# Autodesk Inventor assembly: cradleAssembly
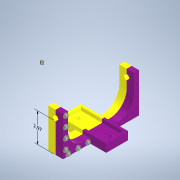
[picture p0: Inventor's stored thumbnail of the model, 180x180]
Saved by Autodesk Inventor 2022 (Build 260153070, 153G)
## iProperties
Created: 2021-06-29
Part Number: cradleAssembly
Document SubType Name: Assembly
Designer: robst
Author: robst
## Documents named in this file (6)
- C:\git\CAD-Development\robSteele\ShapeWays\TelescopeProjects\TelescopeMountNov2020\cradleAssembly.iam
- C:\git\CAD-Development\robSteele\ShapeWays\TelescopeProjects\TelescopeMountNov2020\connectorToTubeBrackeCradlePrintBack.ipt
- C:\git\CAD-Development\robSteele\ShapeWays\TelescopeProjects\TelescopeMountNov2020\connectorToTubeBrackeCradlePrintFront.ipt
- C:\Users\robst\Documents\Inventor\Content Center Files\R2021\en-US\ANSI B18.22.1\ANSI B18.22.1 - No. 10 - Type A.ipt
- C:\Users\robst\Documents\Inventor\Content Center Files\R2021\en-US\ASME B18.21.1(10)\ASME B18.21.1 - No.10(2).ipt
- C:\Users\robst\Documents\Inventor\Content Center Files\R2021\en-US\ANSI B18.6.2(08)\ANSI B18.6.2 - 10-32 UNF - 1.75(17).ipt
## Components (23 placed, 5 different names)
1. connectorToTubeBrackeCradlePrintBack:1 — Mate:1, Flush:1, Flush:2
2. connectorToTubeBrackeCradlePrintFront:1 — Mate:1, Flush:1, Flush:2, Mate:2, Mate:3, Mate:4, Mate:5, Mate:6, Mate:7, Mate:8, Mate:9, Mate:10, Mate:11, Mate:12, Mate:13, Mate:14, Mate:15
3. Plain Washer (Inch) No. 10 - Type A:1 — Mate:2, Mate:3, Insert:1
4. Regular Helical Spring Lock Washer (Inch) No.10:1 — Insert:1, Insert:8
5. Slotted Round Head Cap Screw - Inch No. 10 - 32 - 1 3/4:1 — Insert:8
6. Plain Washer (Inch) No. 10 - Type A:2 — Mate:4, Mate:5, Insert:2
7. Plain Washer (Inch) No. 10 - Type A:3 — Mate:6, Mate:7, Insert:3
8. Plain Washer (Inch) No. 10 - Type A:4 — Mate:8, Mate:9, Insert:4
9. Plain Washer (Inch) No. 10 - Type A:5 — Mate:10, Mate:11, Insert:5
10. Plain Washer (Inch) No. 10 - Type A:6 — Mate:12, Mate:13, Insert:6
11. Plain Washer (Inch) No. 10 - Type A:7 — Mate:14, Mate:15, Insert:7
12. Regular Helical Spring Lock Washer (Inch) No.10:2 — Insert:2, Insert:9
13. Regular Helical Spring Lock Washer (Inch) No.10:3 — Insert:3, Insert:10
14. Regular Helical Spring Lock Washer (Inch) No.10:4 — Insert:4, Insert:11
15. Regular Helical Spring Lock Washer (Inch) No.10:5 — Insert:5, Insert:12
16. Regular Helical Spring Lock Washer (Inch) No.10:6 — Insert:6, Insert:13
17. Regular Helical Spring Lock Washer (Inch) No.10:7 — Insert:7, Insert:14
18. Slotted Round Head Cap Screw - Inch No. 10 - 32 - 1 3/4:2 — Insert:9
19. Slotted Round Head Cap Screw - Inch No. 10 - 32 - 1 3/4:3 — Insert:10
20. Slotted Round Head Cap Screw - Inch No. 10 - 32 - 1 3/4:4 — Insert:11
21. Slotted Round Head Cap Screw - Inch No. 10 - 32 - 1 3/4:5 — Insert:12
22. Slotted Round Head Cap Screw - Inch No. 10 - 32 - 1 3/4:6 — Insert:13
23. Slotted Round Head Cap Screw - Inch No. 10 - 32 - 1 3/4:7 — Insert:14
## Relationships (31: Mate 15, Insert 14, Flush 2)
- Mate:1: connectorToTubeBrackeCradlePrintBack:1 ↔ connectorToTubeBrackeCradlePrintFront:1
- Flush:1: connectorToTubeBrackeCradlePrintBack:1 ↔ connectorToTubeBrackeCradlePrintFront:1
- Flush:2: connectorToTubeBrackeCradlePrintBack:1 ↔ connectorToTubeBrackeCradlePrintFront:1
- Mate:2: connectorToTubeBrackeCradlePrintFront:1 ↔ Plain Washer (Inch) No. 10 - Type A:1
- Mate:3: connectorToTubeBrackeCradlePrintFront:1 ↔ Plain Washer (Inch) No. 10 - Type A:1
- Mate:4: connectorToTubeBrackeCradlePrintFront:1 ↔ Plain Washer (Inch) No. 10 - Type A:2
- Mate:5: connectorToTubeBrackeCradlePrintFront:1 ↔ Plain Washer (Inch) No. 10 - Type A:2
- Mate:6: connectorToTubeBrackeCradlePrintFront:1 ↔ Plain Washer (Inch) No. 10 - Type A:3
- Mate:7: connectorToTubeBrackeCradlePrintFront:1 ↔ Plain Washer (Inch) No. 10 - Type A:3
- Mate:8: connectorToTubeBrackeCradlePrintFront:1 ↔ Plain Washer (Inch) No. 10 - Type A:4
- Mate:9: connectorToTubeBrackeCradlePrintFront:1 ↔ Plain Washer (Inch) No. 10 - Type A:4
- Mate:10: connectorToTubeBrackeCradlePrintFront:1 ↔ Plain Washer (Inch) No. 10 - Type A:5
- Mate:11: connectorToTubeBrackeCradlePrintFront:1 ↔ Plain Washer (Inch) No. 10 - Type A:5
- Mate:12: connectorToTubeBrackeCradlePrintFront:1 ↔ Plain Washer (Inch) No. 10 - Type A:6
- Mate:13: connectorToTubeBrackeCradlePrintFront:1 ↔ Plain Washer (Inch) No. 10 - Type A:6
- Mate:14: connectorToTubeBrackeCradlePrintFront:1 ↔ Plain Washer (Inch) No. 10 - Type A:7
- Mate:15: connectorToTubeBrackeCradlePrintFront:1 ↔ Plain Washer (Inch) No. 10 - Type A:7
- Insert:1: Plain Washer (Inch) No. 10 - Type A:1 ↔ Regular Helical Spring Lock Washer (Inch) No.10:1
- Insert:2: Plain Washer (Inch) No. 10 - Type A:2 ↔ Regular Helical Spring Lock Washer (Inch) No.10:2
- Insert:3: Plain Washer (Inch) No. 10 - Type A:3 ↔ Regular Helical Spring Lock Washer (Inch) No.10:3
- Insert:4: Plain Washer (Inch) No. 10 - Type A:4 ↔ Regular Helical Spring Lock Washer (Inch) No.10:4
- Insert:5: Plain Washer (Inch) No. 10 - Type A:5 ↔ Regular Helical Spring Lock Washer (Inch) No.10:5
- Insert:6: Plain Washer (Inch) No. 10 - Type A:6 ↔ Regular Helical Spring Lock Washer (Inch) No.10:6
- Insert:7: Plain Washer (Inch) No. 10 - Type A:7 ↔ Regular Helical Spring Lock Washer (Inch) No.10:7
- Insert:8: Regular Helical Spring Lock Washer (Inch) No.10:1 ↔ Slotted Round Head Cap Screw - Inch No. 10 - 32 - 1 3/4:1
- Insert:9: Regular Helical Spring Lock Washer (Inch) No.10:2 ↔ Slotted Round Head Cap Screw - Inch No. 10 - 32 - 1 3/4:2
- Insert:10: Regular Helical Spring Lock Washer (Inch) No.10:3 ↔ Slotted Round Head Cap Screw - Inch No. 10 - 32 - 1 3/4:3
- Insert:11: Regular Helical Spring Lock Washer (Inch) No.10:4 ↔ Slotted Round Head Cap Screw - Inch No. 10 - 32 - 1 3/4:4
- Insert:12: Regular Helical Spring Lock Washer (Inch) No.10:5 ↔ Slotted Round Head Cap Screw - Inch No. 10 - 32 - 1 3/4:5
- Insert:13: Regular Helical Spring Lock Washer (Inch) No.10:6 ↔ Slotted Round Head Cap Screw - Inch No. 10 - 32 - 1 3/4:6
- Insert:14: Regular Helical Spring Lock Washer (Inch) No.10:7 ↔ Slotted Round Head Cap Screw - Inch No. 10 - 32 - 1 3/4:7
